# Autodesk Inventor assembly: NMRtray20v2
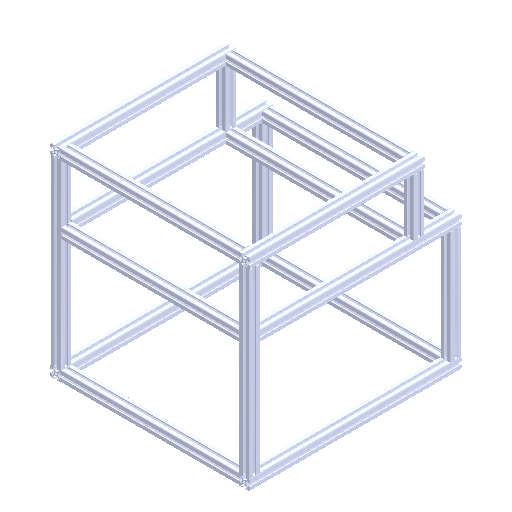
[picture p0: Inventor's stored thumbnail of the model, 512x512]
Saved by Autodesk Inventor 2025 (Build 290162000, 162)
## iProperties
Created: 2025-04-03
Part Number: NMRtray20v2
Description: STEP AP214
Document SubType Name: Assembly
Designer: MK103
Title: NMRtray20v2.STEP
Revision Number: ANY
Sending System: SolidWorks 2024
Preprocessor: SwSTEP 2.0
## Documents named in this file (8)
- C:\Users\mk103\Downloads\NMRCADV20v2.1\NMRCADV20v2.1\NMRtray20v2\NMRtray20v2.iam
- C:\Users\mk103\Downloads\NMRCADV20v2.1\NMRCADV20v2.1\NMRtray20v2\AL409.575_5537T104.ipt
- C:\Users\mk103\Downloads\NMRCADV20v2.1\NMRCADV20v2.1\NMRtray20v2\AL329.575_5537T104.ipt
- C:\Users\mk103\Downloads\NMRCADV20v2.1\NMRCADV20v2.1\NMRtray20v2\AL210_5537T104.ipt
- C:\Users\mk103\Downloads\NMRCADV20v2.1\NMRCADV20v2.1\NMRtray20v2\AL106_5537T104.ipt
- C:\Users\mk103\Downloads\NMRCADV20v2.1\NMRCADV20v2.1\NMRtray20v2\AL325.575_5537T104.ipt
- C:\Users\mk103\Downloads\NMRCADV20v2.1\NMRCADV20v2.1\AL210_5537T104_EDIT.ipt
- C:\Users\mk103\Downloads\NMRCADV20v2.1\NMRCADV20v2.1\AL409.575_5537T104_Edit.ipt
## Components (19 placed, 17 different names)
1. AL409.575_5537T104_1 — Mate:1, Flush:3, Flush:4, Mate:3, Flush:9
2. AL329.575_5537T104_2
3. AL409.575_5537T104_3 — Mate:2, Flush:5, Flush:6, Flush:7, Flush:8
4. AL329.575_5537T104_4 — Mate:3, Flush:8, Flush:9
5. AL210_5537T104_5
6. AL210_5537T104_6
7. AL329.575_5537T104_9 — Mate:4, Flush:11, Flush:12
8. AL329.575_5537T104_11
9. AL325.575_5537T104_14
10. AL106_5537T104_16
11. AL106_5537T104_17
12. AL325.575_5537T104_18
13. AL329.575_5537T104_19
14. AL329.575_5537T104_20
15. AL329.575_5537T104_21
16. AL210_5537T104_EDIT:1 — Mate:1, Flush:3, Flush:4, Flush:13, Flush:14
17. AL210_5537T104_EDIT:2 — Mate:2, Flush:5, Flush:6, Flush:7, Flush:10
18. AL409.575_5537T104_Edit:1 — Flush:10, Mate:4, Flush:11, Flush:12
19. AL409.575_5537T104_Edit:2 — Flush:13, Flush:14
## Relationships (16: Flush 12, Mate 4)
- Mate:1: AL409.575_5537T104_1 ↔ AL210_5537T104_EDIT:1
- Flush:3: AL409.575_5537T104_1 ↔ AL210_5537T104_EDIT:1
- Flush:4: AL409.575_5537T104_1 ↔ AL210_5537T104_EDIT:1
- Mate:2: AL409.575_5537T104_3 ↔ AL210_5537T104_EDIT:2
- Flush:5: AL409.575_5537T104_3 ↔ AL210_5537T104_EDIT:2
- Flush:6: AL409.575_5537T104_3 ↔ AL210_5537T104_EDIT:2
- Flush:7: AL409.575_5537T104_3 ↔ AL210_5537T104_EDIT:2
- Mate:3: AL409.575_5537T104_1 ↔ AL329.575_5537T104_4
- Flush:8: AL409.575_5537T104_3 ↔ AL329.575_5537T104_4
- Flush:9: AL409.575_5537T104_1 ↔ AL329.575_5537T104_4
- Flush:10: AL210_5537T104_EDIT:2 ↔ AL409.575_5537T104_Edit:1
- Mate:4: AL329.575_5537T104_9 ↔ AL409.575_5537T104_Edit:1
- Flush:11: AL329.575_5537T104_9 ↔ AL409.575_5537T104_Edit:1
- Flush:12: AL329.575_5537T104_9 ↔ AL409.575_5537T104_Edit:1
- Flush:13: AL210_5537T104_EDIT:1 ↔ AL409.575_5537T104_Edit:2
- Flush:14: AL210_5537T104_EDIT:1 ↔ AL409.575_5537T104_Edit:2
